# Autodesk Inventor assembly: Chalk Applicator
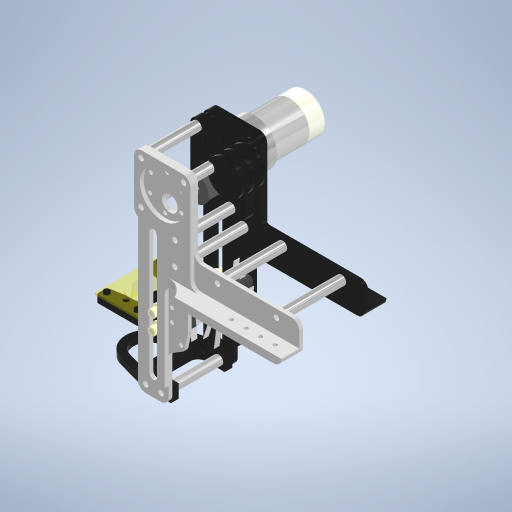
[picture p0: Inventor's stored thumbnail of the model, 512x512]
Saved by Autodesk Inventor 2024 (Build 280153000, 153)
## iProperties
Created: 2023-12-18
Part Number: Chalk Applicator
Document SubType Name: Assembly
Designer: greg
Author: greg
## Documents named in this file (15)
- C:\Users\greg\Documents\Inventor\Capstone\Chalk Applicator\Chalk Applicator.iam
- C:\Users\greg\Documents\Inventor\Capstone\Chalk Applicator\Cross Shaft.iam
- C:\Users\greg\Documents\Inventor\Capstone\Chalk Applicator\Standoff.ipt
- C:\Users\greg\Documents\Inventor\Capstone\Chalk Applicator\Carriage.ipt
- C:\Users\greg\Documents\Inventor\Capstone\Chalk Applicator\Gripper.ipt
- C:\Users\greg\Documents\Inventor\Capstone\Chalk Applicator\Lower Guide.ipt
- C:\Users\greg\Documents\Inventor\Capstone\Chalk Applicator\Side Plate 2.0.ipt
- C:\Users\greg\Documents\Inventor\Capstone\Chalk Applicator\Vince-Motor.ipt
- C:\Users\greg\Documents\Inventor\Capstone\Chalk Applicator\Side Plate 2.0_MIR.ipt
- C:\Users\greg\Documents\Inventor\Capstone\Chalk Applicator\PulleyV2.ipt
- C:\Users\greg\Documents\Inventor\Capstone\Chalk Applicator\Motor Mount Plate.ipt
- C:\Users\greg\Documents\Inventor\Capstone\Chalk Applicator\Standoff-short.ipt
- C:\Users\greg\Documents\Inventor\Capstone\Chalk Applicator\Standoff-short-bottom.ipt
- C:\Users\greg\Documents\Inventor\Capstone\Chalk Applicator\32T GT2 Pulley.ipt
- C:\Users\greg\Documents\Inventor\Capstone\Chalk Applicator\V_153_1C25.ipt
## Components (21 placed, 14 different names)
1. Cross Shaft:1 [sub-assembly] — Mate:29, Tangent:2, Mate:31
2. Cross Shaft:2 [sub-assembly] — Mate:28, Mate:30, Tangent:1, Mate:32
3. Carriage:1 — Mate:28, Mate:29, Mate:30, Insert:11, Insert:12
4. Gripper:1 — Insert:11, Insert:12
5. Lower Guide:1 — Insert:13, Insert:14, Insert:17, Insert:18, Insert:37, Insert:38
6. Side Plate 2.0:1 — Insert:13, Insert:14, Tangent:1, Tangent:2, Mate:31, Mate:32, Insert:23, Insert:25, Insert:26, Insert:27, Insert:28, Insert:39, Tangent:3
7. Side Plate 2.0_MIR:1 — Insert:17, Insert:18, Insert:35, Insert:36, Insert:40, Tangent:4
8. Standoff:7 — Insert:23
9. Standoff:8 — Insert:26
10. Standoff:9 — Insert:25
11. Motor Mount Plate:1 — Insert:27, Insert:28, Insert:29, Insert:30, Insert:31, Insert:32, Insert:33, Insert:34
12. Vince-Motor:1 — Insert:29, Insert:30, Mate:33, Mate:34, Mate:35, Mate:36
13. Standoff-short:1 — Insert:31
14. Standoff-short:2 — Insert:33, Insert:35
15. Standoff-short:3 — Insert:32, Insert:36
16. Standoff-short:4 — Insert:34
17. PulleyV2:1 — Mate:33
18. Standoff-short-bottom:1 — Insert:37, Insert:38
19. 32T GT2 Pulley:1 — Mate:34, Mate:35, Mate:36
20. V_153_1C25:1 — Insert:39, Tangent:3
21. V_153_1C25:2 — Insert:40, Tangent:4
## Relationships (36: Insert 23, Mate 9, Tangent 4)
- Mate:28: Cross Shaft:2 ↔ Carriage:1
- Mate:29: Cross Shaft:1 ↔ Carriage:1
- Mate:30 (1.5875 mm): Cross Shaft:2 ↔ Carriage:1
- Insert:11: Carriage:1 ↔ Gripper:1
- Insert:12: Carriage:1 ↔ Gripper:1
- Insert:13: Lower Guide:1 ↔ Side Plate 2.0:1
- Insert:14: Lower Guide:1 ↔ Side Plate 2.0:1
- Tangent:1: Cross Shaft:2 ↔ Side Plate 2.0:1
- Tangent:2: Cross Shaft:1 ↔ Side Plate 2.0:1
- Mate:31: Cross Shaft:1 ↔ Side Plate 2.0:1
- Mate:32: Cross Shaft:2 ↔ Side Plate 2.0:1
- Insert:17: Lower Guide:1 ↔ Side Plate 2.0_MIR:1
- Insert:18: Lower Guide:1 ↔ Side Plate 2.0_MIR:1
- Insert:23: Side Plate 2.0:1 ↔ Standoff:7
- Insert:25: Side Plate 2.0:1 ↔ Standoff:9
- Insert:26: Side Plate 2.0:1 ↔ Standoff:8
- Insert:27: Side Plate 2.0:1 ↔ Motor Mount Plate:1
- Insert:28: Side Plate 2.0:1 ↔ Motor Mount Plate:1
- Insert:29: Motor Mount Plate:1 ↔ Vince-Motor:1
- Insert:30: Motor Mount Plate:1 ↔ Vince-Motor:1
- Insert:31: Motor Mount Plate:1 ↔ Standoff-short:1
- Insert:32: Motor Mount Plate:1 ↔ Standoff-short:3
- Insert:33: Motor Mount Plate:1 ↔ Standoff-short:2
- Insert:34: Motor Mount Plate:1 ↔ Standoff-short:4
- Insert:35: Side Plate 2.0_MIR:1 ↔ Standoff-short:2
- Insert:36: Side Plate 2.0_MIR:1 ↔ Standoff-short:3
- Mate:33: Vince-Motor:1 ↔ PulleyV2:1
- Insert:37: Lower Guide:1 ↔ Standoff-short-bottom:1
- Insert:38: Lower Guide:1 ↔ Standoff-short-bottom:1
- Mate:34: Vince-Motor:1 ↔ 32T GT2 Pulley:1
- Mate:35: Vince-Motor:1 ↔ 32T GT2 Pulley:1
- Mate:36: Vince-Motor:1 ↔ 32T GT2 Pulley:1
- Insert:39: Side Plate 2.0:1 ↔ V_153_1C25:1
- Tangent:3: Side Plate 2.0:1 ↔ V_153_1C25:1
- Insert:40: Side Plate 2.0_MIR:1 ↔ V_153_1C25:2
- Tangent:4: Side Plate 2.0_MIR:1 ↔ V_153_1C25:2
